# Autodesk Inventor assembly: Structure
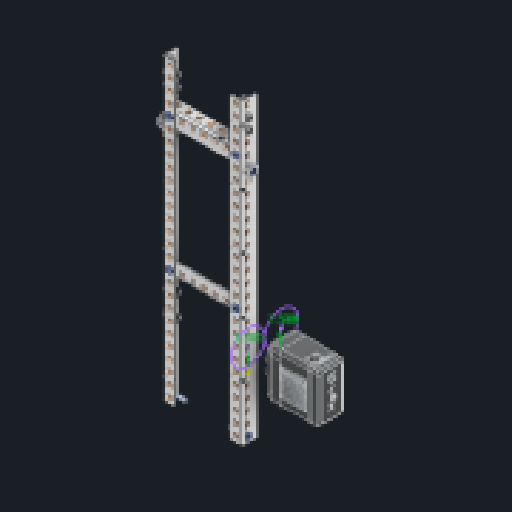
[picture p0: Inventor's stored thumbnail of the model, 512x512]
Saved by Autodesk Inventor 2025 (Build 290162000, 162)
## iProperties
Created: 2024-12-25
Part Number: Structure
Document SubType Name: Assembly
Designer: Averey Ku
Author: Averey Ku
## Documents named in this file (19)
- D:\VEX\High Stakes\CAD\V4\Conveyer\Structure.iam
- D:\VEX\High Stakes\CAD\ROBOPROS-CAD-Inventor\Electronics\Motors with Screws\SteelM-StarS.iam
- D:\VEX\High Stakes\CAD\ROBOPROS-CAD-Inventor\Electronics\Motors with Screws.iam
- D:\VEX\High Stakes\CAD\ROBOPROS-CAD-Inventor\Motion\Shaft LS\Bearing Flat Low Profile.ipt
- D:\VEX\High Stakes\CAD\ROBOPROS-CAD-Inventor\Structure\C Channel\Aluminum 1x3x1 Half Thick Cut\Alu C Half Thick 1x3x1x27.ipt
- D:\VEX\High Stakes\CAD\ROBOPROS-CAD-Inventor\Structure\Hardware\Screw Nylon - Pan Head\NScrew Pan Head Threaded .500.ipt
- D:\VEX\High Stakes\CAD\ROBOPROS-CAD-Inventor\Structure\Hardware\Nut Nylon Thread-Forming.ipt
- D:\VEX\High Stakes\CAD\ROBOPROS-CAD-Inventor\Structure\Hardware\Screw Shoulder Robosource\SScrew Shoulder Smooth .375 x .12.ipt
- D:\VEX\High Stakes\CAD\ROBOPROS-CAD-Inventor\Structure\Hardware\Screw Shoulder Robosource.ipt
- D:\VEX\High Stakes\CAD\ROBOPROS-CAD-Inventor\Structure\Hardware\Nut Nylock.ipt
- D:\VEX\High Stakes\CAD\ROBOPROS-CAD-Inventor\Structure\C Channel\Aluminum 1x3x1 Half Thick Cut\Alu C Half Thick 1x3x1x7.ipt
- D:\VEX\High Stakes\CAD\ROBOPROS-CAD-Inventor\Structure\Hardware\Screw Steel - Star\SScrew Star Smooth .875.ipt
- D:\VEX\High Stakes\CAD\ROBOPROS-CAD-Inventor\Structure\Hardware\Screw Steel - Star.ipt
- D:\VEX\High Stakes\CAD\ROBOPROS-CAD-Inventor\Motion\Spacers\Spacer Nylon .375 OD\NSpacer .375 OD x .500.ipt
- D:\VEX\High Stakes\CAD\ROBOPROS-CAD-Inventor\Motion\Spacers\Spacer Nylon .375 OD.ipt
- D:\VEX\High Stakes\CAD\ROBOPROS-CAD-Inventor\Motion\Spacers\Washer Steel\SWasher .375 OD x .015625.ipt
- D:\VEX\High Stakes\CAD\ROBOPROS-CAD-Inventor\Motion\Spacers\Washer Steel.ipt
- D:\VEX\High Stakes\CAD\ROBOPROS-CAD-Inventor\Structure\1-Post Hex Nut Retainer With Hardware.iam
- D:\VEX\High Stakes\CAD\V4\Conveyer\Custom Parts\Ramp.ipt
## Components (38 placed, 13 different names)
1. Alu C Half Thick 1x3x1x27:1 — Mate:6, Mate:7, Mate:8, Insert:1, Mate:9, Insert:2, Insert:3, Insert:6, Insert:8, Insert:9, Insert:10, Insert:21, Insert:28, Insert:31, Insert:34, Mate:17, Insert:36, Mate:19
2. Bearing Flat Low Profile:3 — Insert:1, Mate:9, Insert:4, Insert:5
3. NScrew Pan Head Threaded .500:1 — Insert:3
4. NScrew Pan Head Threaded .500:2 — Insert:2
5. Nut Nylon Thread-Forming:1 — Insert:5
6. Nut Nylon Thread-Forming:2 — Insert:4
7. SScrew Shoulder Smooth .375 x .12:1 — Insert:6, Mate:14
8. Nut Nylock:1 — Insert:8
9. SScrew Shoulder Smooth .375 x .12:2 — Insert:9
10. Nut Nylock:2 — Insert:10
11. Alu C Half Thick 1x3x1x27:2 — Mate:11, Mate:12, Mate:13, Insert:11, Insert:12, Insert:13, Insert:16, Insert:17, Insert:18, Insert:19, Insert:20, Flush:1, Insert:24, Mate:16, Insert:26, Insert:27, Insert:29, Insert:33, Insert:35, Mate:18, Insert:37, Insert:38, Mate:20
12. Bearing Flat Low Profile:4 — Mate:13, Insert:11, Insert:14, Insert:15
13. NScrew Pan Head Threaded .500:3 — Insert:12
14. NScrew Pan Head Threaded .500:4 — Insert:13
15. Nut Nylon Thread-Forming:3 — Insert:14
16. Nut Nylon Thread-Forming:4 — Insert:15
17. SScrew Shoulder Smooth .375 x .12:3 — Insert:16
18. Nut Nylock:3 — Insert:17
19. SScrew Shoulder Smooth .375 x .12:4 — Insert:18, Mate:15
20. Nut Nylock:4 — Insert:19
21. Alu C Half Thick 1x3x1x7:1 — Insert:21, Mate:15
22. Alu C Half Thick 1x3x1x7:2 — Insert:20, Mate:14
23. Bearing Flat Low Profile:5 — Insert:24, Mate:16, Insert:25
24. NScrew Pan Head Threaded .500:5 — Insert:27
25. NScrew Pan Head Threaded .500:6 — Insert:26
26. Nut Nylon Thread-Forming:5 — Insert:25
27. Nut Nylon Thread-Forming:6
28. SScrew Star Smooth .875:1 — Insert:28
29. SScrew Star Smooth .875:2 — Insert:29
30. NSpacer .375 OD x .500:1 — Insert:30, Insert:31
31. SWasher .375 OD x .015625:1 — Insert:30
32. NSpacer .375 OD x .500:2 — Insert:33
33. SWasher .375 OD x .015625:2
34. 1-Post Hex Nut Retainer With Hardware:1 [sub-assembly] — Insert:34, Mate:17
35. 1-Post Hex Nut Retainer With Hardware:2 [sub-assembly] — Insert:35, Mate:18
36. Ramp:1 — Insert:36, Mate:19, Mate:21, Insert:39
37. Ramp:2 — Insert:37, Insert:38, Mate:20
38. SteelM-StarS:1 [sub-assembly] — Mate:21, Insert:39
## Relationships (53: Insert 37, Mate 15, Flush 1)
- Mate:6 (-171.45 mm): Alu C Half Thick 1x3x1x27:1
- Mate:7 (31.75 mm): Alu C Half Thick 1x3x1x27:1
- Mate:8: Alu C Half Thick 1x3x1x27:1
- Insert:1: Alu C Half Thick 1x3x1x27:1 ↔ Bearing Flat Low Profile:3
- Mate:9: Alu C Half Thick 1x3x1x27:1 ↔ Bearing Flat Low Profile:3
- Insert:2: Alu C Half Thick 1x3x1x27:1 ↔ NScrew Pan Head Threaded .500:2
- Insert:3: Alu C Half Thick 1x3x1x27:1 ↔ NScrew Pan Head Threaded .500:1
- Insert:4 (1.27 mm): Bearing Flat Low Profile:3 ↔ Nut Nylon Thread-Forming:2
- Insert:5 (1.27 mm): Bearing Flat Low Profile:3 ↔ Nut Nylon Thread-Forming:1
- Insert:6: Alu C Half Thick 1x3x1x27:1 ↔ SScrew Shoulder Smooth .375 x .12:1
- Insert:8 (1.5875 mm): Alu C Half Thick 1x3x1x27:1 ↔ Nut Nylock:1
- Insert:9: Alu C Half Thick 1x3x1x27:1 ↔ SScrew Shoulder Smooth .375 x .12:2
- Insert:10 (1.5875 mm): Alu C Half Thick 1x3x1x27:1 ↔ Nut Nylock:2
- Mate:11: Alu C Half Thick 1x3x1x27:2
- Mate:12 (-171.45 mm): Alu C Half Thick 1x3x1x27:2
- Mate:13: Alu C Half Thick 1x3x1x27:2 ↔ Bearing Flat Low Profile:4
- Insert:11: Alu C Half Thick 1x3x1x27:2 ↔ Bearing Flat Low Profile:4
- Insert:12: Alu C Half Thick 1x3x1x27:2 ↔ NScrew Pan Head Threaded .500:3
- Insert:13: Alu C Half Thick 1x3x1x27:2 ↔ NScrew Pan Head Threaded .500:4
- Insert:14 (1.27 mm): Bearing Flat Low Profile:4 ↔ Nut Nylon Thread-Forming:3
- Insert:15 (1.27 mm): Bearing Flat Low Profile:4 ↔ Nut Nylon Thread-Forming:4
- Insert:16: Alu C Half Thick 1x3x1x27:2 ↔ SScrew Shoulder Smooth .375 x .12:3
- Insert:17 (1.5875 mm): Alu C Half Thick 1x3x1x27:2 ↔ Nut Nylock:3
- Insert:18: Alu C Half Thick 1x3x1x27:2 ↔ SScrew Shoulder Smooth .375 x .12:4
- Insert:19 (1.5875 mm): Alu C Half Thick 1x3x1x27:2 ↔ Nut Nylock:4
- Insert:20: Alu C Half Thick 1x3x1x27:2 ↔ Alu C Half Thick 1x3x1x7:2
- Mate:14: SScrew Shoulder Smooth .375 x .12:1 ↔ Alu C Half Thick 1x3x1x7:2
- Flush:1 (31.75 mm): Alu C Half Thick 1x3x1x27:2
- Insert:21: Alu C Half Thick 1x3x1x27:1 ↔ Alu C Half Thick 1x3x1x7:1
- Mate:15: SScrew Shoulder Smooth .375 x .12:4 ↔ Alu C Half Thick 1x3x1x7:1
- [Insert] (1.27 mm): Bearing Flat Low Profile:5 ↔ Nut Nylon Thread-Forming:6
- Insert:24: Alu C Half Thick 1x3x1x27:2 ↔ Bearing Flat Low Profile:5
- Mate:16: Alu C Half Thick 1x3x1x27:2 ↔ Bearing Flat Low Profile:5
- Insert:25 (1.27 mm): Bearing Flat Low Profile:5 ↔ Nut Nylon Thread-Forming:5
- Insert:26: Alu C Half Thick 1x3x1x27:2 ↔ NScrew Pan Head Threaded .500:6
- Insert:27: Alu C Half Thick 1x3x1x27:2 ↔ NScrew Pan Head Threaded .500:5
- Insert:28: Alu C Half Thick 1x3x1x27:1 ↔ SScrew Star Smooth .875:1
- Insert:29: Alu C Half Thick 1x3x1x27:2 ↔ SScrew Star Smooth .875:2
- Insert:30: NSpacer .375 OD x .500:1 ↔ SWasher .375 OD x .015625:1
- Insert:31: Alu C Half Thick 1x3x1x27:1 ↔ NSpacer .375 OD x .500:1
- [Insert]: NSpacer .375 OD x .500:2 ↔ SWasher .375 OD x .015625:2
- Insert:33: Alu C Half Thick 1x3x1x27:2 ↔ NSpacer .375 OD x .500:2
- Insert:34: Alu C Half Thick 1x3x1x27:1 ↔ 1-Post Hex Nut Retainer With Hardware:1
- Mate:17: Alu C Half Thick 1x3x1x27:1 ↔ 1-Post Hex Nut Retainer With Hardware:1
- Insert:35: Alu C Half Thick 1x3x1x27:2 ↔ 1-Post Hex Nut Retainer With Hardware:2
- Mate:18: Alu C Half Thick 1x3x1x27:2 ↔ 1-Post Hex Nut Retainer With Hardware:2
- Insert:36: Alu C Half Thick 1x3x1x27:1 ↔ Ramp:1
- Insert:37: Alu C Half Thick 1x3x1x27:2 ↔ Ramp:2
- Mate:19: Alu C Half Thick 1x3x1x27:1 ↔ Ramp:1
- Insert:38: Alu C Half Thick 1x3x1x27:2 ↔ Ramp:2
- Mate:20: Alu C Half Thick 1x3x1x27:2 ↔ Ramp:2
- Mate:21: Ramp:1 ↔ SteelM-StarS:1
- Insert:39: Ramp:1 ↔ SteelM-StarS:1
## Named parameters: d47_d36 = 1.27 mm, d57_d55 = 0 mm
